# Autodesk Inventor assembly: Motor Bracket
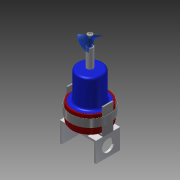
[picture p0: Inventor's stored thumbnail of the model, 180x180]
Saved by Autodesk Inventor 2013 (Build 170138000, 138)
## iProperties
Created: 2014-07-18
Part Number: Motor Bracket
Document SubType Name: Assembly
Designer: Kyle
Author: Kyle
## Documents named in this file (10)
- C:\Users\Kyle\Documents\Autodesk\Inventor\Projects\ROV\Motor Assembly\Motor Bracket.iam
- C:\Users\Kyle\Documents\Autodesk\Inventor\Projects\ROV\Motor Assembly\Mount.ipt
- C:\Users\Kyle\Documents\Autodesk\Inventor\Projects\ROV\Motor Assembly\Plate.ipt
- C:\Users\Kyle\Documents\Autodesk\Inventor\Projects\ROV\Motor Assembly\L Bracket.ipt
- C:\Users\Kyle\Documents\Autodesk\Inventor\Projects\ROV\Motor Assembly\.125 Rivet.ipt
- C:\Users\Kyle\Documents\Autodesk\Inventor\Projects\ROV\Motor\Lg Motor.iam
- C:\Users\Kyle\Documents\Autodesk\Inventor\Projects\ROV\Motor Assembly\Hose Clamp.ipt
- C:\Users\Kyle\Documents\Autodesk\Inventor\Projects\ROV\Motor Assembly\Coupling Bushing.ipt
- C:\Users\Kyle\Documents\Autodesk\Inventor\Projects\ROV\Motor Assembly\Main Prop.ipt
- C:\Users\Kyle\Documents\Autodesk\Inventor\Projects\ROV\Motor Assembly\Prop Screw.ipt
## Components (14 placed, 9 different names)
1. Mount:1 — Mate:1, Mate:2, Mate:3, Mate:4, Angle:1, Mate:5, Mate:6, Angle:2, Mate:7, Mate:8, Mate:9, Tangent:4, Mate:20
2. Plate:1 — Mate:1, Mate:2, Mate:3, Mate:11, Mate:13, Mate:14, Mate:15, Mate:16, Mate:17, Mate:18, Tangent:3
3. L Bracket:1 — Mate:4, Angle:1, Mate:5, Mate:10, Tangent:1
4. L Bracket:2 — Mate:6, Angle:2, Mate:7, Mate:12, Tangent:2
5. .125 Rivet:1 — Mate:11, Mate:15
6. .125 Rivet:2 — Mate:13, Mate:17
7. .125 Rivet:3 — Mate:12, Mate:16
8. .125 Rivet:4 — Mate:10, Mate:14
9. .125 Rivet:5 — Mate:8, Mate:9
10. Lg Motor:1 [sub-assembly] — Mate:18, Tangent:1, Tangent:2, Tangent:3, Tangent:4, Mate:19, Mate:21, Angle:3, Angle:4, Mate:25
11. Hose Clamp:1 — Mate:19, Mate:20
12. Coupling Bushing:1 — Mate:21, Angle:3, Mate:24, Mate:25, Mate:26
13. Main Prop:1 — Mate:24, Angle:4, Mate:26, Mate:27, Mate:28, Mate:29
14. Prop Screw:1 — Mate:27, Mate:28, Mate:29
## Relationships (35: Mate 27, Angle 4, Tangent 4)
- Mate:1: Mount:1 ↔ Plate:1
- Mate:2: Mount:1 ↔ Plate:1
- Mate:3: Mount:1 ↔ Plate:1
- Mate:4: Mount:1 ↔ L Bracket:1
- Angle:1 (0 deg): Mount:1 ↔ L Bracket:1
- Mate:5: Mount:1 ↔ L Bracket:1
- Mate:6: Mount:1 ↔ L Bracket:2
- Angle:2 (0 deg): Mount:1 ↔ L Bracket:2
- Mate:7: Mount:1 ↔ L Bracket:2
- Mate:8: Mount:1 ↔ .125 Rivet:5
- Mate:9: Mount:1 ↔ .125 Rivet:5
- Mate:10: L Bracket:1 ↔ .125 Rivet:4
- Mate:11: Plate:1 ↔ .125 Rivet:1
- Mate:12: L Bracket:2 ↔ .125 Rivet:3
- Mate:13: Plate:1 ↔ .125 Rivet:2
- Mate:14: Plate:1 ↔ .125 Rivet:4
- Mate:15: Plate:1 ↔ .125 Rivet:1
- Mate:16: Plate:1 ↔ .125 Rivet:3
- Mate:17: Plate:1 ↔ .125 Rivet:2
- Mate:18: Plate:1 ↔ Lg Motor:1
- Tangent:1 (-1.905 mm): L Bracket:1 ↔ Lg Motor:1
- Tangent:2 (-1.905 mm): L Bracket:2 ↔ Lg Motor:1
- Tangent:3 (-9.525 mm): Plate:1 ↔ Lg Motor:1
- Tangent:4 (-9.525 mm): Mount:1 ↔ Lg Motor:1
- Mate:19: Lg Motor:1 ↔ Hose Clamp:1
- Mate:20 (15.24 mm): Mount:1 ↔ Hose Clamp:1
- Mate:21: Lg Motor:1 ↔ Coupling Bushing:1
- Angle:3 (180 deg): Lg Motor:1 ↔ Coupling Bushing:1
- Mate:24: Coupling Bushing:1 ↔ Main Prop:1
- Angle:4 (0 deg): Lg Motor:1 ↔ Main Prop:1
- Mate:25: Lg Motor:1 ↔ Coupling Bushing:1
- Mate:26: Coupling Bushing:1 ↔ Main Prop:1
- Mate:27: Main Prop:1 ↔ Prop Screw:1
- Mate:28: Main Prop:1 ↔ Prop Screw:1
- Mate:29: Main Prop:1 ↔ Prop Screw:1
